# Autodesk Inventor assembly: Drive in a Day Frame 2013
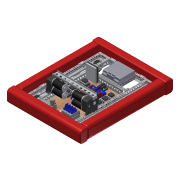
[picture p0: Inventor's stored thumbnail of the model, 180x180]
Saved by Autodesk Inventor 2013 (Build 170138000, 138)
## iProperties
Created: 2013-05-20
Part Number: Drive in a Day Frame 2013
Document SubType Name: Assembly
Designer: Nemo
Mass: 49957.6 g
Surface Area: 54777.3 cm^2
Volume: 51368.1 cm^3
Density: 0.972541 g/cm^3
Author: Nemo
## Documents named in this file (22)
- H:\Nemo\Documents\Robotics\COTS Parts\Drive in a Day\Drive in a Day Frame 2013.iam
- H:\Nemo\Documents\Robotics\COTS Parts\Drive in a Day\217-2593-002 Rev3 Front-Back.ipt
- H:\Nemo\Documents\Robotics\COTS Parts\Drive in a Day\217-2593-001 Rev3 Side Rail.ipt
- H:\Nemo\Documents\Robotics\COTS Parts\Drive in a Day\VersaWheel 2 sprockets for Drive in a Day 2013.iam
- H:\Nemo\Documents\Robotics\COTS Parts\Drive in a Day\DiaD Front Bumper.iam
- H:\Nemo\Documents\Robotics\COTS Parts\Drive in a Day\DiaD Side Bumper.iam
- H:\Nemo\Documents\Robotics\COTS Parts\Drive in a Day\VersaWheel 2 sprockets center wheel for Drive in a Day 2013.iam
- H:\Nemo\Documents\Robotics\COTS Parts\Gearboxes\VexPro Ballshifter 2 stage.iam
- H:\Nemo\Documents\Robotics\COTS Parts\Gearboxes\Components\Ballshifter\Ball Shifter Mounting Bracket.ipt
- H:\Nemo\Documents\Robotics\COTS Parts\Drive in a Day\Custom Ballshifter Cross Brace.ipt
- H:\Nemo\Documents\Robotics\COTS Parts\Drive in a Day\BellyPan for Drive in a Day.ipt
- H:\Nemo\Documents\Robotics\COTS Parts\Electrical - Controls\Battery - FRC 12V.ipt
- H:\Nemo\Documents\Robotics\COTS Parts\Drive in a Day\Drive in a Day Battery Mount.ipt
- H:\Nemo\Documents\Robotics\COTS Parts\Drive in a Day\217-2593-018 Rev1.ipt
- H:\Nemo\Documents\Robotics\COTS Parts\Electrical - Controls\Power Distribution Board.ipt
- H:\Nemo\Documents\Robotics\COTS Parts\Electrical - Controls\120 Amp Breaker - Bussman.ipt
- H:\Nemo\Documents\Robotics\COTS Parts\Electrical - Controls\Talon Controller.ipt
- H:\Nemo\Documents\Robotics\COTS Parts\Electrical - Controls\Viair Compressor.ipt
- H:\Nemo\Documents\Robotics\COTS Parts\Electrical - Controls\cRio FRC II with 3 modules 2 breakouts.ipt
- H:\Nemo\Documents\Robotics\COTS Parts\Electrical - Controls\D-Link Wireless Bridge Radio.ipt
- H:\Nemo\Documents\Robotics\COTS Parts\Electrical - Controls\Digital Sidecar.ipt
- H:\Nemo\Documents\Robotics\COTS Parts\Electrical - Controls\Spike Relay.ipt
## Components (40 placed, 25 different names)
1. 217-2593-002 Rev3 Front — Flush:1, Mate:1, Mate:2, Flush:2, Insert:1, Flush:5, Mate:31
2. 217-2593-002 Rev3 Back — Flush:1, Mate:1, Mate:3, Mate:4, Insert:10, Mate:15, Insert:14, Mate:32
3. 217-2593-001 Rev3 Left outside — Mate:2, Flush:2, Mate:3, Mate:8, Flush:4, Flush:6, Mate:9, Mate:10, Insert:3, Insert:4, Insert:13, Mate:16
4. 217-2593-001 Rev3 Left inside — Mate:8, Flush:4, Mate:10, Mate:24, Angle:3, Mate:25, Mate:36, Mate:51
5. 217-2593-001 Rev3 Right outside — Insert:1, Mate:4, Flush:3, Mate:7, Mate:11, Insert:5, Insert:6, Insert:7
6. 217-2593-001 Rev3 Right inside — Flush:3, Mate:7, Mate:11, Mate:20, Mate:26, Mate:30
7. VersaWheel 2 sprockets for Drive in a Day 2013:2 [sub-assembly] — Insert:4, Flush:10
8. VersaWheel 2 sprockets for Drive in a Day 2013:3 [sub-assembly] — Insert:3
9. VersaWheel 2 sprockets for Drive in a Day 2013:4 [sub-assembly] — Insert:6
10. VersaWheel 2 sprockets for Drive in a Day 2013:5 [sub-assembly] — Insert:7
11. VersaWheel 2 sprockets for Drive in a Day 2013:6 [sub-assembly] — Insert:5
12. DiaD Front Bumper:1 [sub-assembly] — Angle:4, Angle:5
13. DiaD Front Bumper:2 [sub-assembly] — Insert:10, Mate:15
14. DiaD Side Bumper:1 [sub-assembly]
15. DiaD Side Bumper:2 [sub-assembly] — Insert:13, Mate:16
16. VersaWheel 2 sprockets center wheel for Drive in a Day 2013:1 [sub-assembly] — Flush:10
17. VexPro Ballshifter 2 stage:1 [sub-assembly] — Mate:17, Mate:18, Mate:19, Flush:11, Mate:27, Mate:28, Mate:29
18. Ball Shifter Mounting Bracket:1 — Mate:17, Mate:18, Mate:19, Mate:20, Mate:26
19. VexPro Ballshifter 2 stage:2 [sub-assembly] — Mate:21, Mate:22, Mate:23, Flush:11
20. Ball Shifter Mounting Bracket:2 — Mate:21, Mate:22, Mate:23, Mate:24, Angle:3, Mate:25
21. Custom Ballshifter Cross Brace:1 — Mate:27, Mate:28, Mate:29
22. BellyPan for Drive in a Day:1 — Mate:30, Mate:31, Flush:12, Mate:38, Mate:39, Mate:40, Mate:41, Mate:42, Mate:43, Mate:44, Mate:45, Mate:46, Mate:47, Mate:48, Mate:49, Mate:52, Mate:53, Mate:55
23. Battery - FRC 12V:1 — Mate:33, Mate:34, Mate:35
24. Drive in a Day Battery Mount:1 — Insert:14, Mate:32, Mate:33, Mate:34, Mate:35, Mate:37
25. 217-2593-018 Rev1:1 — Mate:36, Flush:13, Mate:37, Mate:50
26. Power Distribution Board:1 — Mate:38, Mate:14
27. 120 Amp Breaker - Bussman:1 — Mate:39
28. Talon Controller:1 — Mate:44, Flush:14, Flush:15, Flush:16
29. Talon Controller:2 — Mate:47, Flush:16
30. Talon Controller:3 — Mate:46, Flush:15
31. Talon Controller:4 — Mate:45, Flush:14
32. Talon Controller:5 — Mate:43, Flush:19
33. Talon Controller:6 — Mate:42, Flush:18
34. Talon Controller:7 — Mate:41, Flush:17
35. Talon Controller:8 — Mate:40, Flush:17, Flush:18, Flush:19
36. Viair Compressor:1 — Mate:48, Angle:4
37. cRio FRC II with 3 modules 2 breakouts:1 — Mate:49, Angle:5, Mate:54
38. D-Link Wireless Bridge Radio:1 — Mate:50, Mate:51, Mate:52
39. Digital Sidecar:1 — Mate:53, Mate:54
40. Spike Relay:1 — Mate:55
## Relationships (90: Mate 53, Flush 19, Insert 13, Angle 5)
- Flush:1: 217-2593-002 Rev3 Front ↔ 217-2593-002 Rev3 Back
- Mate:1: 217-2593-002 Rev3 Front ↔ 217-2593-002 Rev3 Back
- Mate:2: 217-2593-002 Rev3 Front ↔ 217-2593-001 Rev3 Left outside
- Flush:2: 217-2593-002 Rev3 Front ↔ 217-2593-001 Rev3 Left outside
- Mate:3: 217-2593-002 Rev3 Back ↔ 217-2593-001 Rev3 Left outside
- Insert:1: 217-2593-002 Rev3 Front ↔ 217-2593-001 Rev3 Right outside
- Mate:4: 217-2593-002 Rev3 Back ↔ 217-2593-001 Rev3 Right outside
- Flush:3: 217-2593-001 Rev3 Right outside ↔ 217-2593-001 Rev3 Right inside
- Mate:7: 217-2593-001 Rev3 Right outside ↔ 217-2593-001 Rev3 Right inside
- Mate:8: 217-2593-001 Rev3 Left outside ↔ 217-2593-001 Rev3 Left inside
- Flush:4: 217-2593-001 Rev3 Left outside ↔ 217-2593-001 Rev3 Left inside
- Flush:5: 217-2593-002 Rev3 Front
- Flush:6: 217-2593-001 Rev3 Left outside
- Mate:9 (43.815 mm): 217-2593-001 Rev3 Left outside
- Mate:10 (63.5 mm): 217-2593-001 Rev3 Left outside ↔ 217-2593-001 Rev3 Left inside
- Mate:11 (63.5 mm): 217-2593-001 Rev3 Right outside ↔ 217-2593-001 Rev3 Right inside
- Insert:3: 217-2593-001 Rev3 Left outside ↔ VersaWheel 2 sprockets for Drive in a Day 2013:3
- Insert:4: 217-2593-001 Rev3 Left outside ↔ VersaWheel 2 sprockets for Drive in a Day 2013:2
- Insert:5: 217-2593-001 Rev3 Right outside ↔ VersaWheel 2 sprockets for Drive in a Day 2013:6
- Insert:6: 217-2593-001 Rev3 Right outside ↔ VersaWheel 2 sprockets for Drive in a Day 2013:4
- Insert:7: 217-2593-001 Rev3 Right outside ↔ VersaWheel 2 sprockets for Drive in a Day 2013:5
- [Insert]: 217-2593-002 Rev3 Front ↔ DiaD Front Bumper:1
- [Mate]: 217-2593-002 Rev3 Front ↔ DiaD Front Bumper:1
- [Insert]: 217-2593-002 Rev3 Front ↔ DiaD Front Bumper:1
- [Flush]: 217-2593-002 Rev3 Front ↔ DiaD Front Bumper:1
- [Mate] (57.15 mm): DiaD Front Bumper:1
- Insert:10: 217-2593-002 Rev3 Back ↔ DiaD Front Bumper:2
- Mate:15: 217-2593-002 Rev3 Back ↔ DiaD Front Bumper:2
- [Insert]: 217-2593-001 Rev3 Right outside ↔ DiaD Side Bumper:1
- [Angle] (0 deg): 217-2593-001 Rev3 Right outside ↔ DiaD Side Bumper:1
- [Insert]: 217-2593-001 Rev3 Right outside ↔ DiaD Side Bumper:1
- [Angle] (0 deg): 217-2593-001 Rev3 Right outside ↔ DiaD Side Bumper:1
- [Flush]: DiaD Front Bumper:1 ↔ DiaD Side Bumper:1
- [Flush]: 217-2593-001 Rev3 Right outside ↔ DiaD Side Bumper:1
- Insert:13: 217-2593-001 Rev3 Left outside ↔ DiaD Side Bumper:2
- Mate:16: 217-2593-001 Rev3 Left outside ↔ DiaD Side Bumper:2
- Flush:10: VersaWheel 2 sprockets for Drive in a Day 2013:2 ↔ VersaWheel 2 sprockets center wheel for Drive in a Day 2013:1
- Mate:17: VexPro Ballshifter 2 stage:1 ↔ Ball Shifter Mounting Bracket:1
- Mate:18: VexPro Ballshifter 2 stage:1 ↔ Ball Shifter Mounting Bracket:1
- Mate:19: VexPro Ballshifter 2 stage:1 ↔ Ball Shifter Mounting Bracket:1
- Mate:20: 217-2593-001 Rev3 Right inside ↔ Ball Shifter Mounting Bracket:1
- Mate:21: VexPro Ballshifter 2 stage:2 ↔ Ball Shifter Mounting Bracket:2
- Mate:22: VexPro Ballshifter 2 stage:2 ↔ Ball Shifter Mounting Bracket:2
- Mate:23: VexPro Ballshifter 2 stage:2 ↔ Ball Shifter Mounting Bracket:2
- Mate:24: 217-2593-001 Rev3 Left inside ↔ Ball Shifter Mounting Bracket:2
- Angle:3 (0 deg): 217-2593-001 Rev3 Left inside ↔ Ball Shifter Mounting Bracket:2
- Flush:11: VexPro Ballshifter 2 stage:1 ↔ VexPro Ballshifter 2 stage:2
- Mate:25: 217-2593-001 Rev3 Left inside ↔ Ball Shifter Mounting Bracket:2
- Mate:26: 217-2593-001 Rev3 Right inside ↔ Ball Shifter Mounting Bracket:1
- Mate:27: VexPro Ballshifter 2 stage:1 ↔ Custom Ballshifter Cross Brace:1
- Mate:28: VexPro Ballshifter 2 stage:1 ↔ Custom Ballshifter Cross Brace:1
- Mate:29: VexPro Ballshifter 2 stage:1 ↔ Custom Ballshifter Cross Brace:1
- Mate:30: 217-2593-001 Rev3 Right inside ↔ BellyPan for Drive in a Day:1
- Mate:31: 217-2593-002 Rev3 Front ↔ BellyPan for Drive in a Day:1
- Flush:12: BellyPan for Drive in a Day:1
- Insert:14: 217-2593-002 Rev3 Back ↔ Drive in a Day Battery Mount:1
- Mate:32: 217-2593-002 Rev3 Back ↔ Drive in a Day Battery Mount:1
- Mate:33: Battery - FRC 12V:1 ↔ Drive in a Day Battery Mount:1
- Mate:34: Battery - FRC 12V:1 ↔ Drive in a Day Battery Mount:1
- Mate:35: Battery - FRC 12V:1 ↔ Drive in a Day Battery Mount:1
- Mate:36: 217-2593-001 Rev3 Left inside ↔ 217-2593-018 Rev1:1
- Flush:13: 217-2593-018 Rev1:1
- Mate:37 (1.3208 mm): Drive in a Day Battery Mount:1 ↔ 217-2593-018 Rev1:1
- Mate:38: BellyPan for Drive in a Day:1 ↔ Power Distribution Board:1
- Mate:14: Power Distribution Board:1
- Mate:39: BellyPan for Drive in a Day:1 ↔ 120 Amp Breaker - Bussman:1
- Mate:40: BellyPan for Drive in a Day:1 ↔ Talon Controller:8
- Mate:41: BellyPan for Drive in a Day:1 ↔ Talon Controller:7
- Mate:42: BellyPan for Drive in a Day:1 ↔ Talon Controller:6
- Mate:43: BellyPan for Drive in a Day:1 ↔ Talon Controller:5
- Mate:44: BellyPan for Drive in a Day:1 ↔ Talon Controller:1
- Mate:45: BellyPan for Drive in a Day:1 ↔ Talon Controller:4
- Mate:46: BellyPan for Drive in a Day:1 ↔ Talon Controller:3
- Mate:47: BellyPan for Drive in a Day:1 ↔ Talon Controller:2
- Flush:14: Talon Controller:1 ↔ Talon Controller:4
- Flush:15: Talon Controller:1 ↔ Talon Controller:3
- Flush:16: Talon Controller:1 ↔ Talon Controller:2
- Flush:17: Talon Controller:7 ↔ Talon Controller:8
- Flush:18: Talon Controller:6 ↔ Talon Controller:8
- Flush:19: Talon Controller:5 ↔ Talon Controller:8
- Mate:48: BellyPan for Drive in a Day:1 ↔ Viair Compressor:1
- Angle:4 (0 deg): DiaD Front Bumper:1 ↔ Viair Compressor:1
- Mate:49: BellyPan for Drive in a Day:1 ↔ cRio FRC II with 3 modules 2 breakouts:1
- Angle:5 (0 deg): DiaD Front Bumper:1 ↔ cRio FRC II with 3 modules 2 breakouts:1
- Mate:50: 217-2593-018 Rev1:1 ↔ D-Link Wireless Bridge Radio:1
- Mate:51: 217-2593-001 Rev3 Left inside ↔ D-Link Wireless Bridge Radio:1
- Mate:52: BellyPan for Drive in a Day:1 ↔ D-Link Wireless Bridge Radio:1
- Mate:53: BellyPan for Drive in a Day:1 ↔ Digital Sidecar:1
- Mate:54: cRio FRC II with 3 modules 2 breakouts:1 ↔ Digital Sidecar:1
- Mate:55: BellyPan for Drive in a Day:1 ↔ Spike Relay:1
